# Autodesk Inventor assembly: Track Design 9-3-19
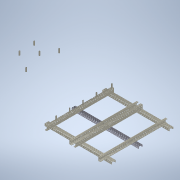
[picture p0: Inventor's stored thumbnail of the model, 180x180]
Saved by Autodesk Inventor 2020 (Build 240168000, 168)
## iProperties
Created: 2019-07-25
Part Number: Track Design 9-3-19
Document SubType Name: Assembly
Designer: Corey
Author: Corey
## Documents named in this file (4)
- C:\Users\spenc\Google Drive\2019_2020 Tower Takeover\CAD\Track Design 1.iam
- C:\Users\spenc\Google Drive\2019_2020 Tower Takeover\CAD\Parts\Structure\C-Channels\Aluminum\2-Wide\Aluminum C-Channel 1x2x1x35.ipt
- C:\Users\spenc\Google Drive\2019_2020 Tower Takeover\CAD\Parts\Structure\C-Channels\Steel\2-Wide\C-Channel 1x2x1x35.ipt
- C:\Users\spenc\Google Drive\2019_2020 Tower Takeover\CAD\Parts\Structure\Standoffs & Couplers\Standoff 1.00''.ipt
## Components (17 placed, 3 different names)
1. Aluminum C-Channel 1x2x1x35:1 — Mate:2, Mate:3, Mate:4, Flush:3, Flush:5, Flush:7, Mate:6, Flush:13, Flush:14, Flush:15, Flush:16, Flush:19
2. Aluminum C-Channel 1x2x1x35:2 — Mate:2, Flush:5, Flush:9, Flush:11, Flush:16, Flush:17, Flush:18
3. Aluminum C-Channel 1x2x1x35:3 — Mate:6, Flush:13, Flush:14
4. Aluminum C-Channel 1x2x1x35:4 — Mate:3, Flush:3, Mate:5, Flush:15
5. Aluminum C-Channel 1x2x1x35:5 — Mate:4, Flush:7, Flush:19, Insert:1, Insert:2, Insert:3, Insert:4, Insert:5
6. Aluminum C-Channel 1x2x1x35:6 — Mate:5, Flush:9, Flush:18
7. C-Channel 1x2x1x35:1 — Flush:11, Flush:17
8. Standoff 1.00'':1
9. Standoff 1.00'':2 — Insert:5
10. Standoff 1.00'':3
11. Standoff 1.00'':4
12. Standoff 1.00'':5 — Insert:1
13. Standoff 1.00'':6 — Insert:3
14. Standoff 1.00'':7 — Insert:2
15. Standoff 1.00'':8 — Insert:4
16. Standoff 1.00'':9
17. Standoff 1.00'':10
## Relationships (22: Flush 12, Mate 5, Insert 5)
- Mate:2: Aluminum C-Channel 1x2x1x35:1 ↔ Aluminum C-Channel 1x2x1x35:2
- Mate:3: Aluminum C-Channel 1x2x1x35:1 ↔ Aluminum C-Channel 1x2x1x35:4
- Mate:4: Aluminum C-Channel 1x2x1x35:1 ↔ Aluminum C-Channel 1x2x1x35:5
- Flush:3: Aluminum C-Channel 1x2x1x35:1 ↔ Aluminum C-Channel 1x2x1x35:4
- Flush:5: Aluminum C-Channel 1x2x1x35:1 ↔ Aluminum C-Channel 1x2x1x35:2
- Flush:7: Aluminum C-Channel 1x2x1x35:1 ↔ Aluminum C-Channel 1x2x1x35:5
- Mate:5: Aluminum C-Channel 1x2x1x35:4 ↔ Aluminum C-Channel 1x2x1x35:6
- Flush:9: Aluminum C-Channel 1x2x1x35:2 ↔ Aluminum C-Channel 1x2x1x35:6
- Flush:11: Aluminum C-Channel 1x2x1x35:2 ↔ C-Channel 1x2x1x35:1
- Mate:6: Aluminum C-Channel 1x2x1x35:1 ↔ Aluminum C-Channel 1x2x1x35:3
- Flush:13: Aluminum C-Channel 1x2x1x35:1 ↔ Aluminum C-Channel 1x2x1x35:3
- Flush:14: Aluminum C-Channel 1x2x1x35:1 ↔ Aluminum C-Channel 1x2x1x35:3
- Flush:15: Aluminum C-Channel 1x2x1x35:1 ↔ Aluminum C-Channel 1x2x1x35:4
- Flush:16: Aluminum C-Channel 1x2x1x35:1 ↔ Aluminum C-Channel 1x2x1x35:2
- Flush:17: Aluminum C-Channel 1x2x1x35:2 ↔ C-Channel 1x2x1x35:1
- Flush:18: Aluminum C-Channel 1x2x1x35:2 ↔ Aluminum C-Channel 1x2x1x35:6
- Flush:19: Aluminum C-Channel 1x2x1x35:1 ↔ Aluminum C-Channel 1x2x1x35:5
- Insert:1: Aluminum C-Channel 1x2x1x35:5 ↔ Standoff 1.00'':5
- Insert:2: Aluminum C-Channel 1x2x1x35:5 ↔ Standoff 1.00'':7
- Insert:3: Aluminum C-Channel 1x2x1x35:5 ↔ Standoff 1.00'':6
- Insert:4: Aluminum C-Channel 1x2x1x35:5 ↔ Standoff 1.00'':8
- Insert:5: Aluminum C-Channel 1x2x1x35:5 ↔ Standoff 1.00'':2
